# Autodesk Inventor assembly: CubSat Assembly
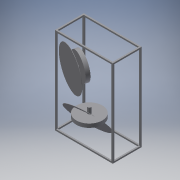
[picture p0: Inventor's stored thumbnail of the model, 180x180]
Saved by Autodesk Inventor 2016 (Build 200138000, 138)
## iProperties
Created: 2015-12-21
Part Number: CubSat Assembly
Document SubType Name: Assembly
Designer: jonathan
Author: jonathan
## Documents named in this file (4)
- C:\Users\jonathan\Dropbox\Satellite\CAD\CubSat Assembly.iam
- C:\Users\jonathan\Dropbox\Satellite\CAD\CubeSat Frame.ipt
- C:\Users\jonathan\Dropbox\Satellite\CAD\Spinning Platform.ipt
- C:\Users\jonathan\Dropbox\Satellite\CAD\Motor Assembly.iam
## Components (5 placed, 3 different names)
1. CubeSat Frame:1
2. Spinning Platform:1
3. Spinning Platform:2 — Mate:1, Rotational:1
4. Motor Assembly:1 [sub-assembly] — Mate:1, Rotational:1
5. Motor Assembly:2 [sub-assembly]
## Relationships (2: Mate 1, RevoluteJoint 1)
- Mate:1: Spinning Platform:2 ↔ Motor Assembly:1
- Rotational:1 [RevoluteJoint]: Spinning Platform:2 ↔ Motor Assembly:1
